# Autodesk Inventor assembly: Assembly Senstable
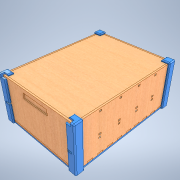
[picture p0: Inventor's stored thumbnail of the model, 180x180]
Saved by Autodesk Inventor 2021 (Build 250183000, 183)
## iProperties
Created: 2021-03-11
Part Number: Assembly Senstable
Document SubType Name: Assembly
Designer: ZiweZhang
Author: ZiweZhang
## Documents named in this file (12)
- E:\School\Projecten\Project 78 - Senstable\Design\Inventor\SensorDoosje\Assembly Senstable.iam
- Assembly SensorDoosje.iam
- E:\School\Projecten\Project 78 - Senstable\Design\Inventor\SensorDoosje\DoosjeOnderkant.ipt
- E:\School\Projecten\Project 78 - Senstable\Design\Inventor\SensorDoosje\DoosjeVoorkant.ipt
- E:\School\Projecten\Project 78 - Senstable\Design\Inventor\SensorDoosje\DoosjeRechter-Linkerkant.ipt
- E:\School\Projecten\Project 78 - Senstable\Design\Inventor\SensorDoosje\DoosjeHoeken.ipt
- E:\School\Projecten\Project 78 - Senstable\Design\Inventor\SensorDoosje\DoosjeGrid.ipt
- E:\School\Projecten\Project 78 - Senstable\Design\Inventor\SensorDoosje\steun.ipt
- E:\School\Projecten\Project 78 - Senstable\Design\Inventor\SensorDoosje\DoosjeHoekenVoorLinks.ipt
- E:\School\Projecten\Project 78 - Senstable\Design\Inventor\SensorDoosje\DoosjeAchterkant.ipt
- E:\School\Projecten\Project 78 - Senstable\Design\Inventor\SensorDoosje\DoosjeHoekenVoorRechts.ipt
- E:\School\Projecten\Project 78 - Senstable\Design\Inventor\SensorDoosje\DoosjeBovenkant.ipt
## Components (17 placed, 8 different names)
1. DoosjeBovenkant:1
2. DoosjeOnderkant:1 — Rigid:1, Rigid:7, Rigid:8, Rigid:10
3. DoosjeAchterkant:1 — Rigid:2, Rigid:5, Rigid:8
4. DoosjeVoorkant:2
5. DoosjeRechter-Linkerkant:1 — Rigid:7, Rigid:9, Rigid:12, Rigid:13, Rigid:14
6. DoosjeRechter-Linkerkant:2 — Rigid:10, Rigid:11, Rigid:15, Rigid:16, Rigid:17
7. DoosjeGrid:1 — Rigid:1
8. DoosjeHoeken:1 — Rigid:5
9. DoosjeHoeken:2 — Rigid:2
10. DoosjeHoeken:3 — Rigid:9
11. DoosjeHoeken:4 — Rigid:11
12. steun:1 — Rigid:13
13. steun:2 — Rigid:17
14. steun:3 — Rigid:12
15. steun:4 — Rigid:16
16. steun:5 — Rigid:15
17. steun:6 — Rigid:14
## Relationships (14: WeldJoint 14)
- Rigid:1 [WeldJoint]: DoosjeOnderkant:1 ↔ DoosjeGrid:1
- Rigid:2 [WeldJoint]: DoosjeAchterkant:1 ↔ DoosjeHoeken:2
- Rigid:5 [WeldJoint]: DoosjeAchterkant:1 ↔ DoosjeHoeken:1
- Rigid:7 [WeldJoint]: DoosjeOnderkant:1 ↔ DoosjeRechter-Linkerkant:1
- Rigid:8 [WeldJoint]: DoosjeOnderkant:1 ↔ DoosjeAchterkant:1
- Rigid:9 [WeldJoint]: DoosjeRechter-Linkerkant:1 ↔ DoosjeHoeken:3
- Rigid:10 [WeldJoint]: DoosjeOnderkant:1 ↔ DoosjeRechter-Linkerkant:2
- Rigid:11 [WeldJoint]: DoosjeRechter-Linkerkant:2 ↔ DoosjeHoeken:4
- Rigid:12 [WeldJoint]: DoosjeRechter-Linkerkant:1 ↔ steun:3
- Rigid:13 [WeldJoint]: DoosjeRechter-Linkerkant:1 ↔ steun:1
- Rigid:14 [WeldJoint]: DoosjeRechter-Linkerkant:1 ↔ steun:6
- Rigid:15 [WeldJoint]: DoosjeRechter-Linkerkant:2 ↔ steun:5
- Rigid:16 [WeldJoint]: DoosjeRechter-Linkerkant:2 ↔ steun:4
- Rigid:17 [WeldJoint]: DoosjeRechter-Linkerkant:2 ↔ steun:2
